# Autodesk Inventor assembly: dining_table
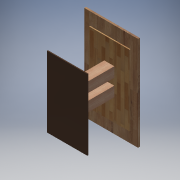
[picture p0: Inventor's stored thumbnail of the model, 180x180]
Saved by Autodesk Inventor 2019 (Build 230136000, 136)
## iProperties
Created: 2019-04-29
Part Number: dining_table
Document SubType Name: Assembly
Designer: Alex
Author: Alex
## Documents named in this file (5)
- P:\Alex\Git\3d_models\dining_table\dining_table.iam
- P:\Alex\Git\3d_models\dining_table\adapter.ipt
- P:\Alex\Git\3d_models\dining_table\baseplate.ipt
- P:\Alex\Git\3d_models\dining_table\stand.ipt
- P:\Alex\Git\3d_models\dining_table\tabletop.ipt
## Components (5 placed, 4 different names)
1. adapter:1 — Mate:3, Flush:3, Mate:5, Flush:4
2. baseplate:1 — Mate:1, Mate:2, Flush:1, Flush:2, Mate:4
3. stand:1 — Mate:2, Mate:3, Flush:6, Flush:8
4. tabletop:1 — Mate:1, Flush:1, Flush:2, Flush:3, Flush:4, Flush:5, Flush:6, Flush:7, Flush:8
5. stand:2 — Mate:4, Mate:5, Flush:5, Flush:7
## Relationships (13: Flush 8, Mate 5)
- Mate:1: baseplate:1 ↔ tabletop:1
- Mate:2: baseplate:1 ↔ stand:1
- Mate:3: adapter:1 ↔ stand:1
- Flush:1 (-175 mm): baseplate:1 ↔ tabletop:1
- Flush:2 (-100 mm): baseplate:1 ↔ tabletop:1
- Flush:3 (-175 mm): adapter:1 ↔ tabletop:1
- Mate:4: baseplate:1 ↔ stand:2
- Mate:5: adapter:1 ↔ stand:2
- Flush:4 (100 mm): adapter:1 ↔ tabletop:1
- Flush:5 (-500 mm): tabletop:1 ↔ stand:2
- Flush:6 (-500 mm): stand:1 ↔ tabletop:1
- Flush:7 (325 mm): tabletop:1 ↔ stand:2
- Flush:8 (325 mm): stand:1 ↔ tabletop:1
